# Autodesk Inventor assembly: Functioning swerve drive (CIM motor shaft)
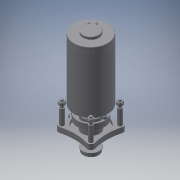
[picture p0: Inventor's stored thumbnail of the model, 180x180]
Saved by Autodesk Inventor 2019 (Build 230136000, 136)
## iProperties
Created: 2019-01-14
Part Number: Functioning swerve drive (CIM motor shaft)
Document SubType Name: Assembly
Designer: josh
Author: josh
## Documents named in this file (5)
- D:\Synthesis Robots\Epsilon\Functioning swerve drive (CIM motor shaft).iam
- D:\Synthesis Robots\Epsilon\FR8ZZ Bearing_smart.ipt
- D:\Synthesis Robots\Epsilon\12T CIM Shaft.ipt
- D:\Synthesis Robots\Epsilon\40T Sleeve Gear REV2.ipt
- D:\Synthesis Robots\Epsilon\VEX 217-2736 0500 Collar Clamp.ipt
## Components (4 placed, 4 different names)
1. FR8ZZ Bearing_smart:2
2. 12T CIM Shaft:2
3. 40T Sleeve Gear REV2:2
4. VEX 217-2736 0500 Collar Clamp:2
## Relationships (3: Mate 3)
- [Mate]: FR8ZZ Bearing_smart:2 ↔ 12T CIM Shaft:2
- [Mate]: FR8ZZ Bearing_smart:2 ↔ 12T CIM Shaft:2
- [Mate]: 12T CIM Shaft:2 ↔ 40T Sleeve Gear REV2:2
## Named parameters: d23_d406_d216 = 0 mm, d24_d189_d93_d166 = 0 mm, d25_d309_d133_d165 = 0 mm
